# Autodesk Inventor assembly: Dome
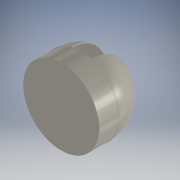
[picture p0: Inventor's stored thumbnail of the model, 180x180]
Saved by Autodesk Inventor 2022 (Build 260153000, 153)
## iProperties
Created: 2021-05-08
Part Number: Dome
Document SubType Name: Assembly
Designer: Mick Veldhuis
Author: Mick Veldhuis
## Documents named in this file (3)
- C:\Users\Mick Veldhuis\Desktop\bsc-project\inventor\observatory\Dome\Dome.iam
- C:\Users\Mick Veldhuis\Desktop\bsc-project\inventor\observatory\Dome\DomeFloor.ipt
- C:\Users\Mick Veldhuis\Desktop\bsc-project\inventor\observatory\Dome\DomeHemisphere.ipt
## Components (2 placed, 2 different names)
1. DomeFloor:1 — DomeAzimuthAxis
2. DomeHemisphere:1 — DomeAzimuthAxis
## Relationships (1: CylindricalJoint 1)
- DomeAzimuthAxis [CylindricalJoint]: DomeFloor:1 ↔ DomeHemisphere:1
